# Autodesk Inventor assembly: Total_new
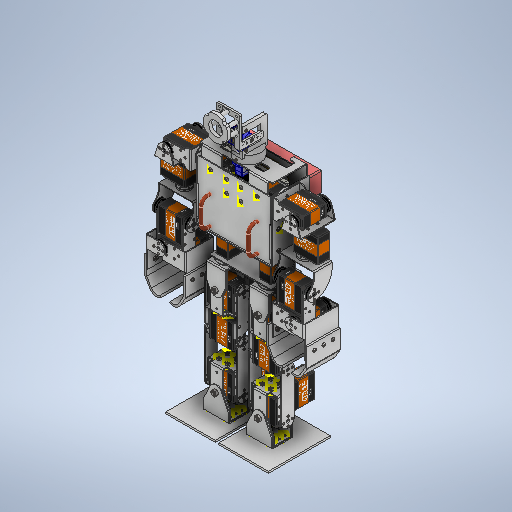
[picture p0: Inventor's stored thumbnail of the model, 512x512]
Saved by Autodesk Inventor 2026.1 (Build 301233000, 233)
## iProperties
Created: 2026-09-27
Part Number: Total_new
Document SubType Name: Assembly
Designer: chris
Author: chris
## Documents named in this file (6)
- C:\Users\chris\Documents\Inventor\RHp_Humanoid_ver1\Total\Total_new.iam
- C:\Users\chris\Documents\Inventor\RHp_Humanoid_ver1\Total\left_Arm.iam
- C:\Users\chris\Documents\Inventor\RHp_Humanoid_ver1\Total\right_Arm.iam
- C:\Users\chris\Documents\Inventor\RHp_Humanoid_ver1\Total\left_leg.iam
- C:\Users\chris\Documents\Inventor\RHp_Humanoid_ver1\Total\right_leg.iam
- C:\Users\chris\Documents\Inventor\RHp_Humanoid_ver1\Total\body_new.iam
## Components (5 placed, 5 different names)
1. body_new:1 [sub-assembly] — Flush:1, Flush:2, Flush:3, Mate:1, Mate:2, Mate:3, Mate:4, Mate:5, Mate:6, Mate:7, Mate:8, Mate:9, Mate:10, Mate:11, Mate:12
2. left_Arm:1 [sub-assembly] — Mate:1, Mate:2, Mate:3
3. right_Arm:1 [sub-assembly] — Mate:4, Mate:5, Mate:6
4. left_leg:1 [sub-assembly] — Mate:10, Mate:11, Mate:12
5. right_leg:1 [sub-assembly] — Mate:7, Mate:8, Mate:9
## Relationships (15: Mate 12, Flush 3)
- Flush:1: body_new:1
- Flush:2: body_new:1
- Flush:3: body_new:1
- Mate:1: body_new:1 ↔ left_Arm:1
- Mate:2: body_new:1 ↔ left_Arm:1
- Mate:3: body_new:1 ↔ left_Arm:1
- Mate:4: body_new:1 ↔ right_Arm:1
- Mate:5: body_new:1 ↔ right_Arm:1
- Mate:6: body_new:1 ↔ right_Arm:1
- Mate:7: body_new:1 ↔ right_leg:1
- Mate:8: body_new:1 ↔ right_leg:1
- Mate:9: body_new:1 ↔ right_leg:1
- Mate:10: body_new:1 ↔ left_leg:1
- Mate:11: body_new:1 ↔ left_leg:1
- Mate:12: body_new:1 ↔ left_leg:1
